# Autodesk Inventor assembly: rocket_assembly
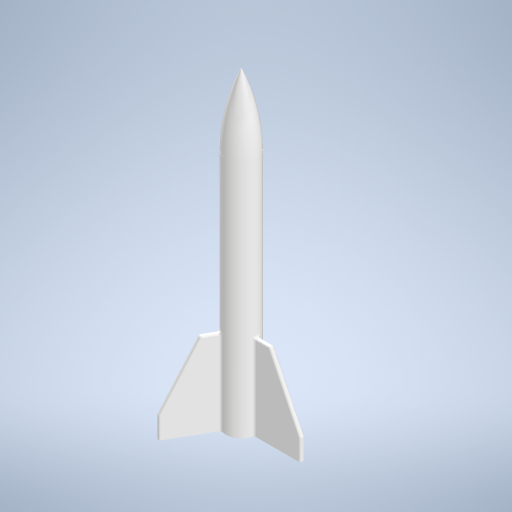
[picture p0: Inventor's stored thumbnail of the model, 512x512]
Saved by Autodesk Inventor 2024 (Build 280153000, 153)
## iProperties
Created: 2024-10-13
Part Number: rocket_assembly
Document SubType Name: Assembly
Designer: soham
Author: soham
## Documents named in this file (3)
- \\Mac\Home\Documents\Inventor\APSS_mech_design\rocket_assembly.iam
- \\Mac\Home\Documents\Inventor\APSS_mech_design\rocket_body.ipt
- \\Mac\Home\Documents\Inventor\APSS_mech_design\rocket_cone.ipt
## Components (2 placed, 2 different names)
1. rocket_body:1 — Rotational:1
2. rocket_cone:1 — Rotational:1
## Relationships (1: RevoluteJoint 1)
- Rotational:1 [RevoluteJoint]: rocket_body:1 ↔ rocket_cone:1
